# Autodesk Inventor assembly: Test_Rig_Assembly
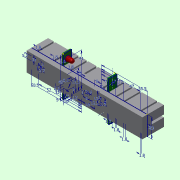
[picture p0: Inventor's stored thumbnail of the model, 180x180]
Saved by Autodesk Inventor 2015 (Build 190159000, 159)
## iProperties
Created: 2015-05-19
Part Number: Test_Rig_Assembly
Document SubType Name: Assembly
Designer: Openlab
Author: Openlab
## Documents named in this file (5)
- D:\Alexey\HS-Spectrophotometer\parts\Test_Rig_Assembly.iam
- D:\Alexey\HS-Spectrophotometer\parts\Distance_test_rig.ipt
- D:\Alexey\HS-Spectrophotometer\parts\Sensor_Board_dummy.ipt
- D:\Alexey\HS-Spectrophotometer\parts\Led_Board_V1.ipt
- D:\Alexey\HS-Spectrophotometer\parts\Cuvette_retainer2.ipt
## Components (5 placed, 4 different names)
1. Distance_test_rig:1 — Mate:1, Mate:2, Mate:3, Mate:4, Mate:5, Mate:6, Mate:7, Mate:8, Mate:9, Mate:10
2. Sensor_Board_dummy:1 — Mate:3, Mate:4
3. Led_Board_V1:1 — Mate:1, Mate:2
4. Cuvette_retainer2:1 — Mate:5, Mate:6, Mate:7
5. Cuvette_retainer2:2 — Mate:8, Mate:9, Mate:10
## Relationships (10: Mate 10)
- Mate:1: Distance_test_rig:1 ↔ Led_Board_V1:1
- Mate:2: Distance_test_rig:1 ↔ Led_Board_V1:1
- Mate:3: Distance_test_rig:1 ↔ Sensor_Board_dummy:1
- Mate:4: Distance_test_rig:1 ↔ Sensor_Board_dummy:1
- Mate:5: Distance_test_rig:1 ↔ Cuvette_retainer2:1
- Mate:6: Distance_test_rig:1 ↔ Cuvette_retainer2:1
- Mate:7: Distance_test_rig:1 ↔ Cuvette_retainer2:1
- Mate:8: Distance_test_rig:1 ↔ Cuvette_retainer2:2
- Mate:9: Distance_test_rig:1 ↔ Cuvette_retainer2:2
- Mate:10: Distance_test_rig:1 ↔ Cuvette_retainer2:2
